# Autodesk Inventor assembly: Zespół1
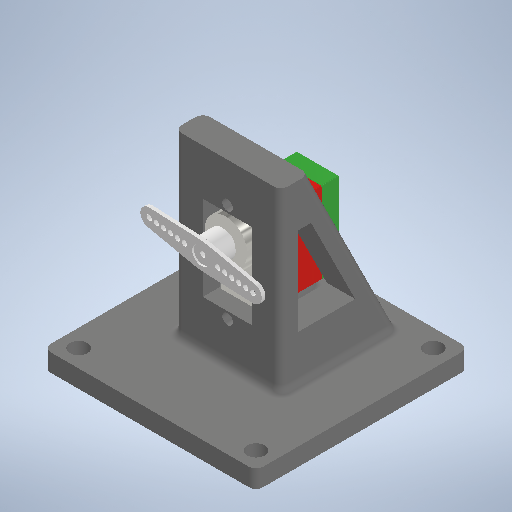
[picture p0: Inventor's stored thumbnail of the model, 512x512]
Saved by Autodesk Inventor 2025.2 (Build 292293000, 293)
## iProperties
Created: 2025-11-25
Part Number: Zespół1
Document SubType Name: Assembly
Designer: juras
Author: juras
## Documents named in this file (3)
- C:\Users\juras\Desktop\AiR SEMESTRY\AiR SEMESTR 5\SYSTEMY MIKROPROCESOROWE\LABORATORIUM\PROJEKT_KULKA_PID\KULKA_PID_KONSTRUKCJA\Zespół1.iam
- C:\Users\juras\Desktop\AiR SEMESTRY\AiR SEMESTR 5\SYSTEMY MIKROPROCESOROWE\LABORATORIUM\PROJEKT_KULKA_PID\KULKA_PID_KONSTRUKCJA\Servo_podstawa.ipt
- C:\Users\juras\Desktop\AiR SEMESTRY\AiR SEMESTR 5\SYSTEMY MIKROPROCESOROWE\LABORATORIUM\PROJEKT_KULKA_PID\KULKA_PID_KONSTRUKCJA\SG90_SG90\SG90_SG90\SG90_SG90.iam
## Components (2 placed, 2 different names)
1. Servo_podstawa:1 — Zestawiające:1, Zestawiające:2, Równoległe:1, Zestawiające:3, Zestawiające:4, Zestawiające:5
2. SG90_SG90:1 [sub-assembly] — Zestawiające:3, Zestawiające:4, Zestawiające:5
## Relationships (6: Mate 5, Flush 1)
- Zestawiające:1 [Mate] (-27.5 mm): Servo_podstawa:1
- Zestawiające:2 [Mate] (-30 mm): Servo_podstawa:1
- Równoległe:1 [Flush] (30 mm): Servo_podstawa:1
- Zestawiające:3 [Mate]: Servo_podstawa:1 ↔ SG90_SG90:1
- Zestawiające:4 [Mate] (1 mm): Servo_podstawa:1 ↔ SG90_SG90:1
- Zestawiające:5 [Mate]: Servo_podstawa:1 ↔ SG90_SG90:1
